# Autodesk Inventor assembly: Arm
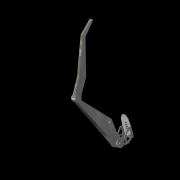
[picture p0: Inventor's stored thumbnail of the model, 180x180]
Saved by Autodesk Inventor 2020 (Build 240168000, 168)
## iProperties
Created: 2020-03-29
Part Number: Arm
Document SubType Name: Assembly
Designer: valer
Mass: 1832.31 g
Surface Area: 2274.86 cm^2
Volume: 1832.31 cm^3
Density: 1 g/cm^3
Author: valer
## Documents named in this file (5)
- C:\Users\valer\Desktop\drummingrobot\src\Arm.iam
- C:\Users\valer\Desktop\drummingrobot\src\UpperArm.ipt
- C:\Users\valer\Desktop\drummingrobot\src\UpperArmBracket.ipt
- C:\Users\valer\Desktop\drummingrobot\src\UpperArmMount.ipt
- C:\Users\valer\Desktop\drummingrobot\src\Forearm.ipt
## Components (5 placed, 4 different names)
1. UpperArm:1 — Mate:11, Mate:12, Flush:1, Mate:13
2. UpperArmBracket:1 — Mate:1, Mate:4, Mate:9
3. UpperArmMount:1 — Mate:1, Mate:2, Mate:3, Mate:4, Mate:7, Mate:8, Mate:10
4. Forearm:1 — Flush:1, Mate:13
5. UpperArmBracket:2 — Mate:2, Mate:3, Mate:9, Mate:10, Mate:11, Mate:12
## Relationships (12: Mate 11, Flush 1)
- Mate:1: UpperArmBracket:1 ↔ UpperArmMount:1
- Mate:2: UpperArmMount:1 ↔ UpperArmBracket:2
- Mate:3: UpperArmMount:1 ↔ UpperArmBracket:2
- Mate:4: UpperArmBracket:1 ↔ UpperArmMount:1
- Mate:7: UpperArmMount:1
- Mate:8: UpperArmMount:1
- Mate:9: UpperArmBracket:1 ↔ UpperArmBracket:2
- Mate:10: UpperArmMount:1 ↔ UpperArmBracket:2
- Mate:11: UpperArm:1 ↔ UpperArmBracket:2
- Mate:12: UpperArm:1 ↔ UpperArmBracket:2
- Flush:1: UpperArm:1 ↔ Forearm:1
- Mate:13: UpperArm:1 ↔ Forearm:1
